# Autodesk Inventor assembly: Assembly_Huawei_P20_Microscope
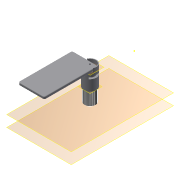
[picture p0: Inventor's stored thumbnail of the model, 180x180]
Saved by Autodesk Inventor 2019 (Build 230136000, 136)
## iProperties
Created: 2019-08-19
Part Number: Assembly_Huawei_P20_Microscope
Document SubType Name: Assembly
Designer: diederichbenedict
Author: diederichbenedict
## Documents named in this file (5)
- C:\Users\diederichbenedict\Dropbox\Dokumente\Promotion\PROJECTS\STORMoChip\INVENTOR\Nanoscopy-on-a-cheap\Assembly_Huawei_P20_Microscope_finite.iam
- C:\Users\diederichbenedict\Dropbox\Dokumente\Promotion\PROJECTS\STORMoChip\INVENTOR\Nanoscopy-on-a-cheap\100_chroma_HQ675_55.ipt
- C:\Users\diederichbenedict\Dropbox\Dokumente\Promotion\PROJECTS\STORMoChip\INVENTOR\Nanoscopy-on-a-cheap\100_Huawei_P9.ipt
- C:\Users\diederichbenedict\Dropbox\Dokumente\Promotion\PROJECTS\STORMoChip\INVENTOR\Nanoscopy-on-a-cheap\00_Microscope_Objective.ipt
- C:\Users\diederichbenedict\Dropbox\Dokumente\Promotion\PROJECTS\STORMoChip\INVENTOR\Nanoscopy-on-a-cheap\10_P9_RMS_Fluofilter.ipt
## Components (4 placed, 4 different names)
1. 100_Huawei_P9:1 — Insert:1, Flush:1
2. 100_chroma_HQ675_55:1 — Insert:1, Insert:2
3. 00_Microscope_Objective:1 — Insert:2, Flush:2
4. 10_P9_RMS_Fluofilter:1 — Flush:1, Flush:2
## Relationships (4: Insert 2, Flush 2)
- Insert:1 (10 mm): 100_Huawei_P9:1 ↔ 100_chroma_HQ675_55:1
- Insert:2 (30 mm): 100_chroma_HQ675_55:1 ↔ 00_Microscope_Objective:1
- Flush:1: 100_Huawei_P9:1 ↔ 10_P9_RMS_Fluofilter:1
- Flush:2: 00_Microscope_Objective:1 ↔ 10_P9_RMS_Fluofilter:1
